# Autodesk Inventor assembly: Mancal com rolamento
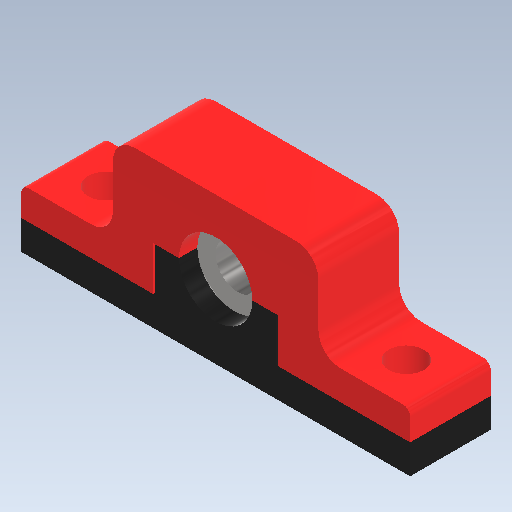
[picture p0: Inventor's stored thumbnail of the model, 512x512]
Saved by Autodesk Inventor 2021 (Build 250183000, 183)
## iProperties
Created: 2021-11-16
Part Number: Mancal com rolamento
Document SubType Name: Assembly
Designer: Mathe
Author: Mathe
## Documents named in this file (4)
- D:\Projetos\Red engrenagens\Mancal com rolamento.iam
- D:\Projetos\Red engrenagens\Mancal superior.ipt
- D:\Projetos\Red engrenagens\Mancal inferior.ipt
- D:\Projetos\Red engrenagens\Rolamento 6x3x2,5mm.ipt
## Components (3 placed, 3 different names)
1. Mancal superior:2 — Mate:1, Mate:2, Mate:3, Flush:1
2. Mancal inferior:1 — Mate:1, Mate:2, Mate:3, Mate:4, Mate:5
3. Rolamento 6x3x2,5mm:1 — Mate:4, Mate:5, Flush:1
## Relationships (6: Mate 5, Flush 1)
- Mate:1: Mancal superior:2 ↔ Mancal inferior:1
- Mate:2: Mancal superior:2 ↔ Mancal inferior:1
- Mate:3: Mancal superior:2 ↔ Mancal inferior:1
- Mate:4: Mancal inferior:1 ↔ Rolamento 6x3x2,5mm:1
- Mate:5: Mancal inferior:1 ↔ Rolamento 6x3x2,5mm:1
- Flush:1: Mancal superior:2 ↔ Rolamento 6x3x2,5mm:1
